# Autodesk Inventor assembly: Мостики
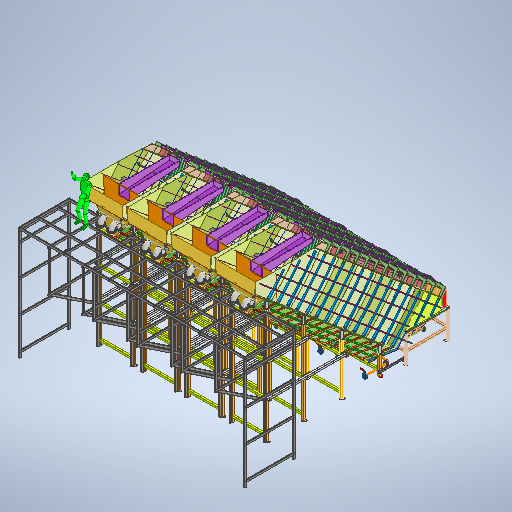
[picture p0: Inventor's stored thumbnail of the model, 512x512]
Saved by Autodesk Inventor 2025 (Build 290162010, 162A)
## iProperties
Created: 2025-01-27
Part Number: Мостики
Document SubType Name: Assembly
Designer: admin
Author: admin
## Documents named in this file (6)
- C:\Users\pokla\Documents\Inventor\Отстойник осветлитель\Manturovo_Se-clar-Gleb\Мостики.iam
- C:\Users\pokla\Documents\Inventor\Отстойник осветлитель\Manturovo_Se-clar-Gleb\ASY MSC 002 отстойник осветлитель.iam
- C:\Users\pokla\Documents\Inventor\Отстойник осветлитель\Manturovo_Se-clar-Gleb\human 01\ч ASY human dummy 01.iam
- C:\Users\pokla\Documents\Inventor\Отстойник осветлитель\Manturovo_Se-clar-Gleb\ASY MSC Платформа отстойников.iam
- C:\Users\pokla\Documents\Inventor\Отстойник осветлитель\Manturovo_Se-clar-Gleb\ASY MSC Опора №1 платф. отст..iam
- C:\Users\pokla\Documents\Inventor\Отстойник осветлитель\Manturovo_Se-clar-Gleb\ASY MSC Опора №2 платф. отст..iam
## Components (16 placed, 5 different names)
1. ASY MSC 002 отстойник осветлитель:1 [sub-assembly] — Flush:1, Flush:2, Flush:3, Flush:4, Rigid:1, Flush:5, Mate:1, Flush:7, Mate:3, Flush:8, Flush:9
2. ASY MSC 002 отстойник осветлитель:2 [sub-assembly] — Rigid:1, Rigid:2
3. ASY MSC 002 отстойник осветлитель:3 [sub-assembly] — Rigid:3
4. ASY MSC 002 отстойник осветлитель:4 [sub-assembly] — Rigid:2, Rigid:3
5. ч ASY human dummy 01:1 [sub-assembly] — Flush:1
6. ASY MSC Платформа отстойников:1 [sub-assembly] — Flush:5, Mate:1, Mate:2, Rigid:4, Rigid:5
7. ASY MSC Опора №1 платф. отст.:1 [sub-assembly] — Rigid:4
8. ASY MSC Опора №1 платф. отст.:2 [sub-assembly] — Rigid:5
9. ASY MSC Опора №2 платф. отст.:2 [sub-assembly] — Rigid:6
10. ASY MSC Опора №2 платф. отст.:1 [sub-assembly] — Flush:7, Mate:3, Flush:8, Flush:9, Rigid:6
11. ASY MSC Опора №2 платф. отст.:3 [sub-assembly]
12. ASY MSC Опора №2 платф. отст.:4 [sub-assembly]
13. ASY MSC Опора №2 платф. отст.:5 [sub-assembly]
14. ASY MSC Опора №2 платф. отст.:6 [sub-assembly]
15. ASY MSC Опора №2 платф. отст.:7 [sub-assembly]
16. ASY MSC Опора №2 платф. отст.:8 [sub-assembly]
## Component patterns: (4 elements, first: ASY MSC Опора №2 платф. отст.:2 + ASY MSC Опора №2 платф. отст.:1)
## Relationships (17: Flush 8, WeldJoint 6, Mate 3)
- Flush:1 (4500 mm): ASY MSC 002 отстойник осветлитель:1 ↔ ч ASY human dummy 01:1
- Flush:2: ASY MSC 002 отстойник осветлитель:1
- Flush:3: ASY MSC 002 отстойник осветлитель:1
- Flush:4: ASY MSC 002 отстойник осветлитель:1
- Rigid:1 [WeldJoint] (50 mm): ASY MSC 002 отстойник осветлитель:1 ↔ ASY MSC 002 отстойник осветлитель:2
- Rigid:2 [WeldJoint] (50 mm): ASY MSC 002 отстойник осветлитель:2 ↔ ASY MSC 002 отстойник осветлитель:4
- Rigid:3 [WeldJoint] (50 mm): ASY MSC 002 отстойник осветлитель:3 ↔ ASY MSC 002 отстойник осветлитель:4
- Flush:5 (-1000 mm): ASY MSC 002 отстойник осветлитель:1 ↔ ASY MSC Платформа отстойников:1
- Mate:1: ASY MSC 002 отстойник осветлитель:1 ↔ ASY MSC Платформа отстойников:1
- Mate:2 (4400 mm): ASY MSC Платформа отстойников:1
- Rigid:4 [WeldJoint]: ASY MSC Платформа отстойников:1 ↔ ASY MSC Опора №1 платф. отст.:1
- Rigid:5 [WeldJoint]: ASY MSC Платформа отстойников:1 ↔ ASY MSC Опора №1 платф. отст.:2
- Flush:7: ASY MSC 002 отстойник осветлитель:1 ↔ ASY MSC Опора №2 платф. отст.:1
- Mate:3: ASY MSC 002 отстойник осветлитель:1 ↔ ASY MSC Опора №2 платф. отст.:1
- Flush:8 (20 mm): ASY MSC 002 отстойник осветлитель:1 ↔ ASY MSC Опора №2 платф. отст.:1
- Flush:9: ASY MSC 002 отстойник осветлитель:1 ↔ ASY MSC Опора №2 платф. отст.:1
- Rigid:6 [WeldJoint] (1305 mm): ASY MSC Опора №2 платф. отст.:2 ↔ ASY MSC Опора №2 платф. отст.:1
